# Autodesk Inventor assembly: 000-dribl-v2
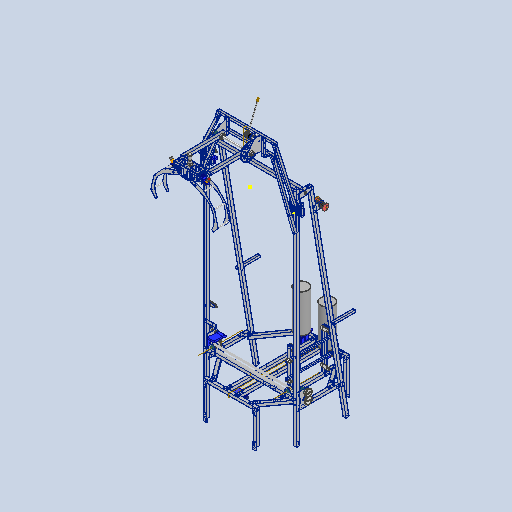
[picture p0: Inventor's stored thumbnail of the model, 512x512]
Saved by Autodesk Inventor 2025.2 (Build 292293000, 293)
## iProperties
Created: 2025-04-03
Part Number: 000-dribl-v2
Document SubType Name: Assembly
Designer: haruy
Author: haruy
## Documents named in this file (63)
- C:\Users\haruy\Documents\ロボコン\NHK2025\cad\nagahisa\dribl\000-dribl-v2.iam
- C:\Users\haruy\Documents\ロボコン\NHK2025\cad\nagahisa\dribl\dribl-v3-Sketch-Base.ipt
- C:\Users\haruy\Documents\ロボコン\NHK2025\cad\nagahisa\dribl\dribl-v1-Plate-5.ipt
- C:\Users\haruy\Documents\ロボコン\NHK2025\cad\nagahisa\dribl\dribl-v1-Plate-3.ipt
- C:\Users\haruy\Documents\ロボコン\NHK2025\cad\nagahisa\dribl\dribl-v1-Plate-4.ipt
- C:\Users\haruy\Documents\ロボコン\NHK2025\cad\nagahisa\dribl\dribl-v3-Plate-1.ipt
- C:\Users\haruy\Documents\ロボコン\NHK2025\cad\nagahisa\dribl\dribl-v3-Plate-2.ipt
- C:\Users\haruy\Documents\ロボコン\NHK2025\cad\nagahisa\dribl\dribl-v3-ASP-arm.ipt
- C:\Users\haruy\Documents\ロボコン\NHK2025\cad\nagahisa\dribl\dribl-v1-Shaft-spesa-57.ipt
- C:\Users\haruy\Documents\ロボコン\NHK2025\cad\nagahisa\dribl\dribl-v1-Plate-8.ipt
- C:\Users\haruy\Documents\ロボコン\NHK2025\cad\000_parts\モーター\robomaster\M2006 P36\RoboMaster M2006 P36\RoboMaster M2006 P36.ipt
- C:\Users\haruy\Documents\ロボコン\NHK2025\cad\nagahisa\dribl\dribl-v3-Plate-6.ipt
- C:\Users\haruy\Documents\ロボコン\NHK2025\cad\nagahisa\dribl\dribl-v3-Plate-7.ipt
- C:\Users\haruy\Documents\ロボコン\NHK2025\cad\nagahisa\dribl\dribl-v3-Plate-8.ipt
- C:\Users\haruy\Documents\ロボコン\NHK2025\cad\nagahisa\dribl\dribl-v3-Plate-9.ipt
- C:\Users\haruy\Documents\ロボコン\NHK2025\cad\nagahisa\dribl\dribl-v3-Plate-10.ipt
- C:\Users\haruy\Documents\ロボコン\NHK2025\cad\nagahisa\dribl\dribl-v3-Plate-11.ipt
- C:\Users\haruy\Documents\ロボコン\NHK2025\cad\nagahisa\dribl\dribl-v3-Plate-12.ipt
- C:\Users\haruy\Documents\ロボコン\NHK2025\cad\nagahisa\dribl\dribl-v1-Plate-14.ipt
- C:\Users\haruy\Documents\ロボコン\NHK2025\cad\nagahisa\dribl\dribl-v1-3DP-P-F.ipt
- C:\Users\haruy\Documents\ロボコン\NHK2025\cad\nagahisa\dribl\roller-Base-v1-petbottle.ipt
- C:\Users\haruy\Documents\ロボコン\NHK2025\cad\nagahisa\dribl\dribl-v3-Plate-13.ipt
- C:\Users\haruy\Documents\ロボコン\NHK2025\cad\nagahisa\dribl\dribl-v3-Plate-14.ipt
- C:\Users\haruy\Documents\ロボコン\NHK2025\cad\nagahisa\base_weel\base_weel-v2-Plate-8.ipt
- C:\Users\haruy\Documents\ロボコン\NHK2025\cad\nagahisa\dribl\dribl-v3-ASP-2.ipt
- C:\Users\haruy\Documents\ロボコン\NHK2025\cad\nagahisa\base_weel\base_weel-v2-POM-pc-F-1.ipt
- C:\Users\haruy\Documents\ロボコン\NHK2025\cad\nagahisa\base_weel\base_weel-v2-POM-pc-F-2.ipt
- C:\Users\haruy\Documents\ロボコン\NHK2025\cad\nagahisa\dribl\dribl-v3-Plate-15.ipt
- C:\Users\haruy\Documents\ロボコン\NHK2025\cad\nagahisa\dribl\dribl-v1-Plate-13.ipt
- C:\Users\haruy\Documents\ロボコン\NHK2025\cad\000_parts\回路関連\EMO\emo_sa.ipt
- C:\Users\haruy\Documents\ロボコン\NHK2025\cad\nagahisa\dribl\dribl-v1-Plate-12.ipt
- C:\Users\haruy\Documents\ロボコン\NHK2025\cad\000_parts\センサー\VX-012-1A3\VX-012-1A3\VX-012-1A3.iam
- C:\Users\haruy\Documents\ロボコン\NHK2025\cad\nagahisa\dribl\R2-Rzvector\TH22_bearing_12_18_19.5_sn.ipt
- C:\Users\haruy\Documents\ロボコン\NHK2025\cad\nagahisa\dribl\SCSNAJ12-16b.ipt
- C:\Users\haruy\Documents\ロボコン\NHK2025\cad\nagahisa\dribl\dribl-v1-Shaft-2.ipt
- C:\Users\haruy\Documents\ロボコン\NHK2025\cad\nagahisa\dribl\dribl-v3-3DP-2.ipt
- C:\Users\haruy\Documents\ロボコン\NHK2025\cad\000_parts\センサー\realsense\D435i_Solid.ipt
- C:\Users\haruy\Documents\ロボコン\NHK2025\cad\nagahisa\dribl\R2-Rzvector\bear_f8_12_sa.ipt
- C:\Users\haruy\Documents\ロボコン\NHK2025\cad\nagahisa\dribl\R2-Rzvector\bear_10_15_sn.ipt
- C:\Users\haruy\Documents\ロボコン\NHK2025\cad\nagahisa\dribl\SCTW12.iam
- C:\Users\haruy\Documents\ロボコン\NHK2025\cad\nagahisa\base_weel\SCSWA8-8.iam
- C:\Users\haruy\Documents\ロボコン\NHK2025\cad\nagahisa\belt_liner\SSCSW10-10b.ipt
- C:\Users\haruy\Documents\ロボコン\NHK2025\cad\nagahisa\dribl\000-dribl-v2\デザイン アクセラレータ\平歯車1.iam
- C:\Users\haruy\Documents\ロボコン\NHK2025\cad\nagahisa\dribl\000-dribl-v2\デザイン アクセラレータ\平歯車2.iam
- C:\Users\haruy\Documents\ロボコン\NHK2025\cad\nagahisa\hand\grab\hand-grab-v5-Plate-6.ipt
- C:\Users\haruy\Documents\ロボコン\NHK2025\cad\nagahisa\hand\grab\hand-grab-v5-Plate-7.ipt
- C:\Users\haruy\Documents\ロボコン\NHK2025\cad\nagahisa\hand\grab\000-hand-grab-v5.iam
- C:\Users\haruy\Documents\ロボコン\NHK2025\cad\nagahisa\hand\grab\hand-grab-v5-ASP-1.ipt
- C:\Users\haruy\Documents\ロボコン\NHK2025\cad\nagahisa\dribl\SCSW12-10.iam
- C:\Users\haruy\Documents\ロボコン\NHK2025\cad\nagahisa\dribl\dribl-v4-Plate-1.ipt
- C:\Users\haruy\Documents\ロボコン\NHK2025\cad\nagahisa\dribl\dribl-v4-Plate-2.ipt
- C:\Users\haruy\Documents\ロボコン\NHK2025\cad\nagahisa\dribl\000-dribl-v2\デザイン アクセラレータ\歯付きベルト伝達2.iam
- C:\Users\haruy\Documents\ロボコン\NHK2025\cad\nagahisa\dribl\000-dribl-v2\デザイン アクセラレータ\平歯車3.iam
- C:\Users\haruy\Documents\ロボコン\NHK2025\cad\nagahisa\dribl\SCSW6-10b.ipt
- C:\Users\haruy\Documents\ロボコン\NHK2025\cad\nagahisa\dribl\dribl-v4-Plate-3.ipt
- C:\Users\haruy\Documents\ロボコン\NHK2025\cad\nagahisa\dribl\R2-Rzvector\RZvector-v1-Plate-B-F.ipt
- C:\Users\haruy\Documents\ロボコン\NHK2025\cad\nagahisa\dribl\dribl-v4-3DP-1.ipt
- C:\Users\haruy\Documents\ロボコン\NHK2025\cad\nagahisa\dribl\dribl-v4-Plate-4.ipt
- C:\Users\haruy\Documents\ロボコン\NHK2025\cad\nagahisa\dribl\dribl-v1-Shaft-4.ipt
- C:\Users\haruy\Documents\ロボコン\NHK2025\cad\nagahisa\dribl\dribl-v1-Shaft-6.ipt
- C:\Users\haruy\Documents\ロボコン\NHK2025\cad\nagahisa\dribl\SMB1_5-20_SMB1_5-20_On.iam
- C:\Users\haruy\Documents\ロボコン\NHK2025\cad\nagahisa\dribl\dribl-v1-Shaft-1.ipt
- C:\Users\haruy\Documents\ロボコン\NHK2025\cad\nagahisa\dribl\dribl-v4-3DP-2.ipt
## Components (125 placed, 60 different names)
1. dribl-v3-Sketch-Base:1 — 挿入:11, 挿入:13, 挿入:14, 挿入:15, 挿入:16, 挿入:17, 挿入:18, 挿入:19, 挿入:20, 挿入:21, 挿入:22, 挿入:23, 挿入:24, 挿入:25, 挿入:26, 挿入:27, 挿入:28, 挿入:29, 挿入:30, 挿入:31, 挿入:32, 挿入:33, 正接:1, 正接:2, 正接:3, 正接:4, 挿入:44, 挿入:45, 挿入:46, 挿入:47, 挿入:48, 挿入:49, 挿入:50, 挿入:51, 挿入:52, 挿入:53, 挿入:56, 挿入:57, 挿入:58, 挿入:59, 挿入:60, 挿入:61, 挿入:62, 挿入:63, 挿入:64, 挿入:65, 挿入:70, 挿入:71, 挿入:72, 挿入:73, 挿入:74, 挿入:75, 挿入:76, 挿入:77, 挿入:78, 挿入:79, 挿入:80, 挿入:81, 挿入:82, 挿入:83, 挿入:84, 挿入:85, 挿入:90, 挿入:91, 挿入:92, 挿入:93, 挿入:94, 挿入:95, 挿入:96, 挿入:97, メイト:4, メイト:6, 挿入:102, 挿入:103, 挿入:104, 挿入:105, 挿入:106, 挿入:107, 挿入:108, 挿入:109, 挿入:128, 挿入:129, 挿入:130, 挿入:131, 挿入:132, 挿入:133, 挿入:134, 挿入:135, フラッシュ:1, 挿入:163, 挿入:164, 挿入:221, 挿入:225, 挿入:233, 挿入:234, 挿入:235, 挿入:236, 挿入:252, 挿入:253, メイト:16, メイト:17, 挿入:254, 挿入:255, 挿入:263, 挿入:264
2. dribl-v1-Plate-5:1 — 挿入:13, 挿入:173, 挿入:175, 挿入:264, 挿入:266, 挿入:267
3. dribl-v1-Plate-5:2 — 挿入:11, 挿入:174, 挿入:176, 挿入:263, 角度:1
4. dribl-v1-Plate-3:1 — 挿入:14, 挿入:15, 挿入:167, 挿入:183
5. dribl-v1-Plate-4:1 — 挿入:16, 挿入:17, 挿入:168
6. dribl-v3-Plate-1:1 — 挿入:18, 挿入:19, 挿入:172
7. dribl-v3-Plate-1:2 — 挿入:20, 挿入:21, 挿入:171
8. dribl-v3-Plate-1:3 — 挿入:22, 挿入:23, 挿入:170
9. dribl-v3-Plate-1:4 — 挿入:24, 挿入:25, 挿入:169
10. dribl-v3-Plate-2:1 — 挿入:26, 挿入:27, 挿入:179
11. dribl-v3-Plate-2:2 — 挿入:28, 挿入:29, 挿入:180
12. dribl-v3-Plate-2:3 — 挿入:32, 挿入:33, 挿入:177
13. dribl-v3-Plate-2:4 — 挿入:30, 挿入:31, 挿入:178
14. dribl-v3-ASP-arm:1 — 正接:1, 正接:2, 正接:3, 正接:4, 挿入:202, 挿入:203, 挿入:204, 挿入:205, 挿入:212, 挿入:213, 挿入:214, 挿入:215, 挿入:216, 挿入:217, 挿入:218, 挿入:219, 挿入:237, 挿入:238, 挿入:239, 挿入:240, 挿入:241, 挿入:268, 挿入:269
15. dribl-v1-Shaft-spesa-57:1 — 挿入:41, 挿入:206
16. dribl-v1-Shaft-spesa-57:2 — 挿入:208
17. dribl-v1-Shaft-spesa-57:3 — 挿入:42, 挿入:207
18. dribl-v1-Plate-8:1 — 挿入:41, 挿入:42, 挿入:43, 挿入:208
19. RoboMaster M2006 P36:1 — 挿入:43, メイト:15
20. dribl-v3-Plate-6:1 — 挿入:44, 挿入:45
21. dribl-v3-Plate-6:2 — 挿入:50, 挿入:51
22. dribl-v3-Plate-6:3 — 挿入:48, 挿入:49
23. dribl-v3-Plate-6:4 — 挿入:46, 挿入:47
24. dribl-v3-Plate-7:1 — 挿入:52, 挿入:53
25. dribl-v3-Plate-7:4 — 挿入:56, 挿入:57
26. dribl-v3-Plate-8:1 — 挿入:58, 挿入:59
27. dribl-v3-Plate-8:2 — 挿入:60, 挿入:61
28. dribl-v3-Plate-9:1 — 挿入:62, 挿入:63
29. dribl-v3-Plate-9:3 — 挿入:64, 挿入:65
30. dribl-v3-Plate-10:1 — 挿入:72, 挿入:73
31. dribl-v3-Plate-10:2 — 挿入:74, 挿入:75
32. dribl-v3-Plate-10:3 — 挿入:70, 挿入:71
33. dribl-v3-Plate-10:4 — 挿入:76, 挿入:77
34. dribl-v3-Plate-11:1 — 挿入:78, 挿入:79
35. dribl-v3-Plate-11:2 — 挿入:82, 挿入:83
36. dribl-v3-Plate-11:3 — 挿入:80, 挿入:81
37. dribl-v3-Plate-11:4 — 挿入:84, 挿入:85
38. dribl-v3-Plate-12:1 — 挿入:90, 挿入:91
39. dribl-v3-Plate-12:2 — 挿入:92, 挿入:93
40. dribl-v1-Plate-14:1 — 挿入:96, 挿入:97
41. dribl-v1-Plate-14:2 — 挿入:94, 挿入:95
42. dribl-v1-3DP-P-F:1 — 挿入:100, メイト:6, メイト:16
43. roller-Base-v1-petbottle:1 — 挿入:100
44. dribl-v1-3DP-P-F:2 — メイト:4, 挿入:101, メイト:17
45. roller-Base-v1-petbottle:2 — 挿入:101
46. dribl-v3-Plate-13:1 — 挿入:102, 挿入:103
47. dribl-v3-Plate-14:1 — 挿入:104, 挿入:105
48. base_weel-v2-Plate-8:1 — 挿入:106, 挿入:107, 挿入:110, 挿入:111
49. base_weel-v2-Plate-8:2 — 挿入:108, 挿入:109
50. dribl-v3-ASP-2:1 — 挿入:110, 挿入:111, 挿入:112, 挿入:113, 挿入:114, 挿入:115, 挿入:116, 挿入:117, 挿入:118, 挿入:119, 挿入:120, 挿入:121, 挿入:122, 挿入:123, 挿入:124, 挿入:125, 挿入:126, 挿入:127
51. base_weel-v2-POM-pc-F-1:1 — 挿入:112, 挿入:113
52. base_weel-v2-POM-pc-F-1:2 — 挿入:114, 挿入:115
53. base_weel-v2-POM-pc-F-2:1 — 挿入:118, 挿入:119
54. base_weel-v2-POM-pc-F-2:2 — 挿入:116, 挿入:117
55. base_weel-v2-POM-pc-F-2:3 — 挿入:122, 挿入:123
56. base_weel-v2-POM-pc-F-2:4 — 挿入:120, 挿入:121
57. base_weel-v2-POM-pc-F-1:3 — 挿入:126, 挿入:127
58. base_weel-v2-POM-pc-F-1:4 — 挿入:124, 挿入:125
59. dribl-v3-Plate-15:1 — 挿入:128, 挿入:129
60. dribl-v3-Plate-15:2 — 挿入:130, 挿入:131
61. dribl-v3-Plate-11:7 — 挿入:132, 挿入:133
62. dribl-v1-Plate-13:1 — 挿入:134, 挿入:135, 挿入:136
63. emo_sa:1 — 挿入:136
64. VX-012-1A3:1 [sub-assembly] — 挿入:223, 挿入:224
65. TH22_bearing_12_18_19.5_sn:1 — 挿入:160, 挿入:210
66. TH22_bearing_12_18_19.5_sn:2 — 挿入:194, 挿入:209
67. SCSNAJ12-16b:1 — 挿入:194
68. SCSNAJ12-16b:2 — 挿入:160, 挿入:195
69. dribl-v1-Shaft-2:1 — 挿入:195, メイト:13
70. dribl-v3-3DP-2:1 — 挿入:163, 挿入:164, 挿入:165, 挿入:166
71. D435i_Solid:1 — 挿入:165, 挿入:166
72. TH22_bearing_12_18_19.5_sn:3 — 挿入:167, 挿入:184
73. TH22_bearing_12_18_19.5_sn:4 — 挿入:168
74. TH22_bearing_12_18_19.5_sn:5 — 挿入:170
75. TH22_bearing_12_18_19.5_sn:6 — 挿入:169, フラッシュ:2
76. TH22_bearing_12_18_19.5_sn:7 — 挿入:171
77. TH22_bearing_12_18_19.5_sn:8 — 挿入:172, 挿入:261
78. TH22_bearing_12_18_19.5_sn:9 — 挿入:173
79. TH22_bearing_12_18_19.5_sn:10 — 挿入:174, 挿入:181
80. bear_f8_12_sa:1 — 挿入:175, 挿入:258
81. bear_f8_12_sa:2 — 挿入:176, 挿入:182
82. bear_10_15_sn:3 — 挿入:178
83. bear_10_15_sn:4 — 挿入:177
84. bear_10_15_sn:5 — 挿入:179
85. bear_10_15_sn:6 — 挿入:180
86. SCTW12:1 [sub-assembly] — 挿入:181, メイト:20
87. SCSWA8-8:1 [sub-assembly] — 挿入:182, メイト:18, メイト:19
88. SSCSW10-10b:1 — 挿入:183, メイト:9
89. SCTW12:2 [sub-assembly] — 挿入:184, メイト:7, メイト:8
90. 平歯車:1 [sub-assembly] — メイト:7, メイト:8, メイト:9
91. 平歯車:2 [sub-assembly] — メイト:18, メイト:19, メイト:20
92. hand-grab-v5-Plate-6:1 — 挿入:202, 挿入:203, 挿入:206, 挿入:207, 挿入:210, 挿入:211
93. hand-grab-v5-Plate-7:1 — 挿入:204, 挿入:205, 挿入:209
94. 000-hand-grab-v5:1 [sub-assembly] — 挿入:196, 挿入:197, 挿入:198, 挿入:199
95. hand-grab-v5-ASP-1:1 — 挿入:196, 挿入:197, 挿入:200
96. hand-grab-v5-ASP-1:2 — 挿入:198, 挿入:199, 挿入:201, 挿入:211, メイト:14
97. SCSW12-10:1 [sub-assembly] — 挿入:201
98. SCSW12-10:2 [sub-assembly] — 挿入:200
99. dribl-v4-Plate-1:1 — 挿入:212, 挿入:213
100. dribl-v4-Plate-1:2 — 挿入:214, 挿入:215
101. dribl-v4-Plate-2:1 — 挿入:216, 挿入:217
102. dribl-v4-Plate-2:2 — 挿入:218, 挿入:219
103. 歯付きベルト伝達:1 [sub-assembly]
104. 平歯車:3 [sub-assembly] — メイト:13, メイト:14, メイト:15, 挿入:220
105. SCSW6-10b:1 — 挿入:220
106. dribl-v1-Plate-12:2 — 挿入:221, 挿入:223, 挿入:224, 挿入:233
107. dribl-v1-Plate-12:3 — 挿入:225, 挿入:227, 挿入:228, 挿入:234
108. VX-012-1A3:3 [sub-assembly] — 挿入:227, 挿入:228
109. dribl-v1-Plate-12:4 — 挿入:231, 挿入:232, 挿入:235, 挿入:236
110. VX-012-1A3:4 [sub-assembly] — 挿入:231, 挿入:232
111. dribl-v4-Plate-3:1 — 挿入:240, 挿入:241, 挿入:242, 挿入:243, 挿入:244, 挿入:245
112. dribl-v4-Plate-3:2 — 挿入:237, 挿入:238, 挿入:239, 挿入:246, 挿入:247, 挿入:248, 挿入:249
113. RZvector-v1-Plate-B-F:1 — 挿入:242, 挿入:243
114. RZvector-v1-Plate-B-F:2 — 挿入:244, 挿入:245
115. RZvector-v1-Plate-B-F:3 — 挿入:246, 挿入:247
116. RZvector-v1-Plate-B-F:4 — 挿入:248, 挿入:249
117. dribl-v4-3DP-1:1 — 挿入:268, 挿入:269
118. dribl-v4-Plate-4:1 — 挿入:252, 挿入:253
119. dribl-v1-Plate-12:5 — 挿入:254, 挿入:255, 挿入:256, 挿入:257
120. VX-012-1A3:5 [sub-assembly] — 挿入:256, 挿入:257
121. dribl-v1-Shaft-4:1 — 挿入:258
122. dribl-v1-Shaft-6:1 — 挿入:265, 角度:1
123. SMB1_5-20_SMB1_5-20_On:1 [sub-assembly] — 挿入:262, 挿入:265
124. dribl-v1-Shaft-1:1 — 挿入:261, 挿入:262
125. dribl-v4-3DP-2:1 — 挿入:266, 挿入:267
## Relationships (217: Insert 197, Mate 13, Tangent 4, Flush 2, Angle 1)
- 挿入:11 [Insert]: dribl-v3-Sketch-Base:1 ↔ dribl-v1-Plate-5:2
- 挿入:13 [Insert]: dribl-v3-Sketch-Base:1 ↔ dribl-v1-Plate-5:1
- 挿入:14 [Insert]: dribl-v3-Sketch-Base:1 ↔ dribl-v1-Plate-3:1
- 挿入:15 [Insert]: dribl-v3-Sketch-Base:1 ↔ dribl-v1-Plate-3:1
- 挿入:16 [Insert]: dribl-v3-Sketch-Base:1 ↔ dribl-v1-Plate-4:1
- 挿入:17 [Insert]: dribl-v3-Sketch-Base:1 ↔ dribl-v1-Plate-4:1
- 挿入:18 [Insert]: dribl-v3-Sketch-Base:1 ↔ dribl-v3-Plate-1:1
- 挿入:19 [Insert]: dribl-v3-Sketch-Base:1 ↔ dribl-v3-Plate-1:1
- 挿入:20 [Insert]: dribl-v3-Sketch-Base:1 ↔ dribl-v3-Plate-1:2
- 挿入:21 [Insert]: dribl-v3-Sketch-Base:1 ↔ dribl-v3-Plate-1:2
- 挿入:22 [Insert]: dribl-v3-Sketch-Base:1 ↔ dribl-v3-Plate-1:3
- 挿入:23 [Insert]: dribl-v3-Sketch-Base:1 ↔ dribl-v3-Plate-1:3
- 挿入:24 [Insert]: dribl-v3-Sketch-Base:1 ↔ dribl-v3-Plate-1:4
- 挿入:25 [Insert]: dribl-v3-Sketch-Base:1 ↔ dribl-v3-Plate-1:4
- 挿入:26 [Insert]: dribl-v3-Sketch-Base:1 ↔ dribl-v3-Plate-2:1
- 挿入:27 [Insert]: dribl-v3-Sketch-Base:1 ↔ dribl-v3-Plate-2:1
- 挿入:28 [Insert]: dribl-v3-Sketch-Base:1 ↔ dribl-v3-Plate-2:2
- 挿入:29 [Insert]: dribl-v3-Sketch-Base:1 ↔ dribl-v3-Plate-2:2
- 挿入:30 [Insert]: dribl-v3-Sketch-Base:1 ↔ dribl-v3-Plate-2:4
- 挿入:31 [Insert]: dribl-v3-Sketch-Base:1 ↔ dribl-v3-Plate-2:4
- 挿入:32 [Insert]: dribl-v3-Sketch-Base:1 ↔ dribl-v3-Plate-2:3
- 挿入:33 [Insert]: dribl-v3-Sketch-Base:1 ↔ dribl-v3-Plate-2:3
- 正接:1 [Tangent]: dribl-v3-Sketch-Base:1 ↔ dribl-v3-ASP-arm:1
- 正接:2 [Tangent]: dribl-v3-Sketch-Base:1 ↔ dribl-v3-ASP-arm:1
- 正接:3 [Tangent]: dribl-v3-Sketch-Base:1 ↔ dribl-v3-ASP-arm:1
- 正接:4 [Tangent]: dribl-v3-Sketch-Base:1 ↔ dribl-v3-ASP-arm:1
- 挿入:41 [Insert]: dribl-v1-Shaft-spesa-57:1 ↔ dribl-v1-Plate-8:1
- 挿入:42 [Insert]: dribl-v1-Shaft-spesa-57:3 ↔ dribl-v1-Plate-8:1
- 挿入:43 [Insert]: dribl-v1-Plate-8:1 ↔ RoboMaster M2006 P36:1
- 挿入:44 [Insert]: dribl-v3-Sketch-Base:1 ↔ dribl-v3-Plate-6:1
- 挿入:45 [Insert]: dribl-v3-Sketch-Base:1 ↔ dribl-v3-Plate-6:1
- 挿入:46 [Insert]: dribl-v3-Sketch-Base:1 ↔ dribl-v3-Plate-6:4
- 挿入:47 [Insert]: dribl-v3-Sketch-Base:1 ↔ dribl-v3-Plate-6:4
- 挿入:48 [Insert]: dribl-v3-Sketch-Base:1 ↔ dribl-v3-Plate-6:3
- 挿入:49 [Insert]: dribl-v3-Sketch-Base:1 ↔ dribl-v3-Plate-6:3
- 挿入:50 [Insert]: dribl-v3-Sketch-Base:1 ↔ dribl-v3-Plate-6:2
- 挿入:51 [Insert]: dribl-v3-Sketch-Base:1 ↔ dribl-v3-Plate-6:2
- 挿入:52 [Insert]: dribl-v3-Sketch-Base:1 ↔ dribl-v3-Plate-7:1
- 挿入:53 [Insert]: dribl-v3-Sketch-Base:1 ↔ dribl-v3-Plate-7:1
- 挿入:56 [Insert]: dribl-v3-Sketch-Base:1 ↔ dribl-v3-Plate-7:4
- 挿入:57 [Insert]: dribl-v3-Sketch-Base:1 ↔ dribl-v3-Plate-7:4
- 挿入:58 [Insert]: dribl-v3-Sketch-Base:1 ↔ dribl-v3-Plate-8:1
- 挿入:59 [Insert]: dribl-v3-Sketch-Base:1 ↔ dribl-v3-Plate-8:1
- 挿入:60 [Insert]: dribl-v3-Sketch-Base:1 ↔ dribl-v3-Plate-8:2
- 挿入:61 [Insert]: dribl-v3-Sketch-Base:1 ↔ dribl-v3-Plate-8:2
- 挿入:62 [Insert]: dribl-v3-Sketch-Base:1 ↔ dribl-v3-Plate-9:1
- 挿入:63 [Insert]: dribl-v3-Sketch-Base:1 ↔ dribl-v3-Plate-9:1
- 挿入:64 [Insert]: dribl-v3-Sketch-Base:1 ↔ dribl-v3-Plate-9:3
- 挿入:65 [Insert]: dribl-v3-Sketch-Base:1 ↔ dribl-v3-Plate-9:3
- 挿入:70 [Insert]: dribl-v3-Sketch-Base:1 ↔ dribl-v3-Plate-10:3
- 挿入:71 [Insert]: dribl-v3-Sketch-Base:1 ↔ dribl-v3-Plate-10:3
- 挿入:72 [Insert]: dribl-v3-Sketch-Base:1 ↔ dribl-v3-Plate-10:1
- 挿入:73 [Insert]: dribl-v3-Sketch-Base:1 ↔ dribl-v3-Plate-10:1
- 挿入:74 [Insert]: dribl-v3-Sketch-Base:1 ↔ dribl-v3-Plate-10:2
- 挿入:75 [Insert]: dribl-v3-Sketch-Base:1 ↔ dribl-v3-Plate-10:2
- 挿入:76 [Insert]: dribl-v3-Sketch-Base:1 ↔ dribl-v3-Plate-10:4
- 挿入:77 [Insert]: dribl-v3-Sketch-Base:1 ↔ dribl-v3-Plate-10:4
- 挿入:78 [Insert]: dribl-v3-Sketch-Base:1 ↔ dribl-v3-Plate-11:1
- 挿入:79 [Insert]: dribl-v3-Sketch-Base:1 ↔ dribl-v3-Plate-11:1
- 挿入:80 [Insert]: dribl-v3-Sketch-Base:1 ↔ dribl-v3-Plate-11:3
- 挿入:81 [Insert]: dribl-v3-Sketch-Base:1 ↔ dribl-v3-Plate-11:3
- 挿入:82 [Insert]: dribl-v3-Sketch-Base:1 ↔ dribl-v3-Plate-11:2
- 挿入:83 [Insert]: dribl-v3-Sketch-Base:1 ↔ dribl-v3-Plate-11:2
- 挿入:84 [Insert]: dribl-v3-Sketch-Base:1 ↔ dribl-v3-Plate-11:4
- 挿入:85 [Insert]: dribl-v3-Sketch-Base:1 ↔ dribl-v3-Plate-11:4
- 挿入:90 [Insert]: dribl-v3-Sketch-Base:1 ↔ dribl-v3-Plate-12:1
- 挿入:91 [Insert]: dribl-v3-Sketch-Base:1 ↔ dribl-v3-Plate-12:1
- 挿入:92 [Insert]: dribl-v3-Sketch-Base:1 ↔ dribl-v3-Plate-12:2
- 挿入:93 [Insert]: dribl-v3-Sketch-Base:1 ↔ dribl-v3-Plate-12:2
- 挿入:94 [Insert]: dribl-v3-Sketch-Base:1 ↔ dribl-v1-Plate-14:2
- 挿入:95 [Insert]: dribl-v3-Sketch-Base:1 ↔ dribl-v1-Plate-14:2
- 挿入:96 [Insert]: dribl-v3-Sketch-Base:1 ↔ dribl-v1-Plate-14:1
- 挿入:97 [Insert]: dribl-v3-Sketch-Base:1 ↔ dribl-v1-Plate-14:1
- 挿入:100 [Insert]: dribl-v1-3DP-P-F:1 ↔ roller-Base-v1-petbottle:1
- メイト:4 [Mate]: dribl-v3-Sketch-Base:1 ↔ dribl-v1-3DP-P-F:2
- 挿入:101 [Insert]: dribl-v1-3DP-P-F:2 ↔ roller-Base-v1-petbottle:2
- メイト:6 [Mate]: dribl-v3-Sketch-Base:1 ↔ dribl-v1-3DP-P-F:1
- 挿入:102 [Insert]: dribl-v3-Sketch-Base:1 ↔ dribl-v3-Plate-13:1
- 挿入:103 [Insert]: dribl-v3-Sketch-Base:1 ↔ dribl-v3-Plate-13:1
- 挿入:104 [Insert]: dribl-v3-Sketch-Base:1 ↔ dribl-v3-Plate-14:1
- 挿入:105 [Insert]: dribl-v3-Sketch-Base:1 ↔ dribl-v3-Plate-14:1
- 挿入:106 [Insert]: dribl-v3-Sketch-Base:1 ↔ base_weel-v2-Plate-8:1
- 挿入:107 [Insert]: dribl-v3-Sketch-Base:1 ↔ base_weel-v2-Plate-8:1
- 挿入:108 [Insert]: dribl-v3-Sketch-Base:1 ↔ base_weel-v2-Plate-8:2
- 挿入:109 [Insert]: dribl-v3-Sketch-Base:1 ↔ base_weel-v2-Plate-8:2
- 挿入:110 [Insert]: base_weel-v2-Plate-8:1 ↔ dribl-v3-ASP-2:1
- 挿入:111 [Insert]: base_weel-v2-Plate-8:1 ↔ dribl-v3-ASP-2:1
- 挿入:112 [Insert]: dribl-v3-ASP-2:1 ↔ base_weel-v2-POM-pc-F-1:1
- 挿入:113 [Insert]: dribl-v3-ASP-2:1 ↔ base_weel-v2-POM-pc-F-1:1
- 挿入:114 [Insert]: dribl-v3-ASP-2:1 ↔ base_weel-v2-POM-pc-F-1:2
- 挿入:115 [Insert]: dribl-v3-ASP-2:1 ↔ base_weel-v2-POM-pc-F-1:2
- 挿入:116 [Insert]: dribl-v3-ASP-2:1 ↔ base_weel-v2-POM-pc-F-2:2
- 挿入:117 [Insert]: dribl-v3-ASP-2:1 ↔ base_weel-v2-POM-pc-F-2:2
- 挿入:118 [Insert]: dribl-v3-ASP-2:1 ↔ base_weel-v2-POM-pc-F-2:1
- 挿入:119 [Insert]: dribl-v3-ASP-2:1 ↔ base_weel-v2-POM-pc-F-2:1
- 挿入:120 [Insert]: dribl-v3-ASP-2:1 ↔ base_weel-v2-POM-pc-F-2:4
- 挿入:121 [Insert]: dribl-v3-ASP-2:1 ↔ base_weel-v2-POM-pc-F-2:4
- 挿入:122 [Insert]: dribl-v3-ASP-2:1 ↔ base_weel-v2-POM-pc-F-2:3
- 挿入:123 [Insert]: dribl-v3-ASP-2:1 ↔ base_weel-v2-POM-pc-F-2:3
- 挿入:124 [Insert]: dribl-v3-ASP-2:1 ↔ base_weel-v2-POM-pc-F-1:4
- 挿入:125 [Insert]: dribl-v3-ASP-2:1 ↔ base_weel-v2-POM-pc-F-1:4
- 挿入:126 [Insert]: dribl-v3-ASP-2:1 ↔ base_weel-v2-POM-pc-F-1:3
- 挿入:127 [Insert]: dribl-v3-ASP-2:1 ↔ base_weel-v2-POM-pc-F-1:3
- 挿入:128 [Insert]: dribl-v3-Sketch-Base:1 ↔ dribl-v3-Plate-15:1
- 挿入:129 [Insert]: dribl-v3-Sketch-Base:1 ↔ dribl-v3-Plate-15:1
- 挿入:130 [Insert]: dribl-v3-Sketch-Base:1 ↔ dribl-v3-Plate-15:2
- 挿入:131 [Insert]: dribl-v3-Sketch-Base:1 ↔ dribl-v3-Plate-15:2
- 挿入:132 [Insert]: dribl-v3-Sketch-Base:1 ↔ dribl-v3-Plate-11:7
- 挿入:133 [Insert]: dribl-v3-Sketch-Base:1 ↔ dribl-v3-Plate-11:7
- 挿入:134 [Insert]: dribl-v3-Sketch-Base:1 ↔ dribl-v1-Plate-13:1
- 挿入:135 [Insert]: dribl-v3-Sketch-Base:1 ↔ dribl-v1-Plate-13:1
- 挿入:136 [Insert]: dribl-v1-Plate-13:1 ↔ emo_sa:1
- フラッシュ:1 [Flush] (-10 mm): dribl-v3-Sketch-Base:1
- 挿入:160 [Insert]: TH22_bearing_12_18_19.5_sn:1 ↔ SCSNAJ12-16b:2
- 挿入:163 [Insert]: dribl-v3-Sketch-Base:1 ↔ dribl-v3-3DP-2:1
- 挿入:164 [Insert]: dribl-v3-Sketch-Base:1 ↔ dribl-v3-3DP-2:1
- 挿入:165 [Insert]: dribl-v3-3DP-2:1 ↔ D435i_Solid:1
- 挿入:166 [Insert]: dribl-v3-3DP-2:1 ↔ D435i_Solid:1
- 挿入:167 [Insert]: dribl-v1-Plate-3:1 ↔ TH22_bearing_12_18_19.5_sn:3
- 挿入:168 [Insert]: dribl-v1-Plate-4:1 ↔ TH22_bearing_12_18_19.5_sn:4
- 挿入:169 [Insert]: dribl-v3-Plate-1:4 ↔ TH22_bearing_12_18_19.5_sn:6
- 挿入:170 [Insert]: dribl-v3-Plate-1:3 ↔ TH22_bearing_12_18_19.5_sn:5
- 挿入:171 [Insert]: dribl-v3-Plate-1:2 ↔ TH22_bearing_12_18_19.5_sn:7
- 挿入:172 [Insert]: dribl-v3-Plate-1:1 ↔ TH22_bearing_12_18_19.5_sn:8
- 挿入:173 [Insert]: dribl-v1-Plate-5:1 ↔ TH22_bearing_12_18_19.5_sn:9
- 挿入:174 [Insert]: dribl-v1-Plate-5:2 ↔ TH22_bearing_12_18_19.5_sn:10
- 挿入:175 [Insert]: dribl-v1-Plate-5:1 ↔ bear_f8_12_sa:1
- 挿入:176 [Insert]: dribl-v1-Plate-5:2 ↔ bear_f8_12_sa:2
- 挿入:177 [Insert]: dribl-v3-Plate-2:3 ↔ bear_10_15_sn:4
- 挿入:178 [Insert]: dribl-v3-Plate-2:4 ↔ bear_10_15_sn:3
- 挿入:179 [Insert]: dribl-v3-Plate-2:1 ↔ bear_10_15_sn:5
- 挿入:180 [Insert]: dribl-v3-Plate-2:2 ↔ bear_10_15_sn:6
- 挿入:181 [Insert] (5 mm): TH22_bearing_12_18_19.5_sn:10 ↔ SCTW12:1
- 挿入:182 [Insert] (9.3 mm): bear_f8_12_sa:2 ↔ SCSWA8-8:1
- 挿入:183 [Insert] (7 mm): dribl-v1-Plate-3:1 ↔ SSCSW10-10b:1
- 挿入:184 [Insert] (4 mm): TH22_bearing_12_18_19.5_sn:3 ↔ SCTW12:2
- メイト:7 [Mate]: SCTW12:2 ↔ 平歯車:1
- メイト:8 [Mate]: SCTW12:2 ↔ 平歯車:1
- メイト:9 [Mate]: SSCSW10-10b:1 ↔ 平歯車:1
- 挿入:194 [Insert]: TH22_bearing_12_18_19.5_sn:2 ↔ SCSNAJ12-16b:1
- 挿入:195 [Insert]: SCSNAJ12-16b:2 ↔ dribl-v1-Shaft-2:1
- 挿入:196 [Insert]: 000-hand-grab-v5:1 ↔ hand-grab-v5-ASP-1:1
- 挿入:197 [Insert]: 000-hand-grab-v5:1 ↔ hand-grab-v5-ASP-1:1
- 挿入:198 [Insert]: 000-hand-grab-v5:1 ↔ hand-grab-v5-ASP-1:2
- 挿入:199 [Insert]: 000-hand-grab-v5:1 ↔ hand-grab-v5-ASP-1:2
- 挿入:200 [Insert]: hand-grab-v5-ASP-1:1 ↔ SCSW12-10:2
- 挿入:201 [Insert]: hand-grab-v5-ASP-1:2 ↔ SCSW12-10:1
- 挿入:202 [Insert]: dribl-v3-ASP-arm:1 ↔ hand-grab-v5-Plate-6:1
- 挿入:203 [Insert]: dribl-v3-ASP-arm:1 ↔ hand-grab-v5-Plate-6:1
- 挿入:204 [Insert]: dribl-v3-ASP-arm:1 ↔ hand-grab-v5-Plate-7:1
- 挿入:205 [Insert]: dribl-v3-ASP-arm:1 ↔ hand-grab-v5-Plate-7:1
- 挿入:206 [Insert]: dribl-v1-Shaft-spesa-57:1 ↔ hand-grab-v5-Plate-6:1
- 挿入:207 [Insert]: dribl-v1-Shaft-spesa-57:3 ↔ hand-grab-v5-Plate-6:1
- 挿入:208 [Insert]: dribl-v1-Shaft-spesa-57:2 ↔ dribl-v1-Plate-8:1
- 挿入:209 [Insert]: TH22_bearing_12_18_19.5_sn:2 ↔ hand-grab-v5-Plate-7:1
- 挿入:210 [Insert]: TH22_bearing_12_18_19.5_sn:1 ↔ hand-grab-v5-Plate-6:1
- 挿入:211 [Insert] (13 mm): hand-grab-v5-Plate-6:1 ↔ hand-grab-v5-ASP-1:2
- 挿入:212 [Insert]: dribl-v3-ASP-arm:1 ↔ dribl-v4-Plate-1:1
- 挿入:213 [Insert]: dribl-v3-ASP-arm:1 ↔ dribl-v4-Plate-1:1
- 挿入:214 [Insert]: dribl-v3-ASP-arm:1 ↔ dribl-v4-Plate-1:2
- 挿入:215 [Insert]: dribl-v3-ASP-arm:1 ↔ dribl-v4-Plate-1:2
- 挿入:216 [Insert]: dribl-v3-ASP-arm:1 ↔ dribl-v4-Plate-2:1
- 挿入:217 [Insert]: dribl-v3-ASP-arm:1 ↔ dribl-v4-Plate-2:1
- 挿入:218 [Insert]: dribl-v3-ASP-arm:1 ↔ dribl-v4-Plate-2:2
- 挿入:219 [Insert]: dribl-v3-ASP-arm:1 ↔ dribl-v4-Plate-2:2
- フラッシュ:2 [Flush] (9 mm): TH22_bearing_12_18_19.5_sn:6
- メイト:13 [Mate]: dribl-v1-Shaft-2:1 ↔ 平歯車:3
- メイト:14 [Mate]: hand-grab-v5-ASP-1:2 ↔ 平歯車:3
- メイト:15 [Mate]: RoboMaster M2006 P36:1 ↔ 平歯車:3
- 挿入:220 [Insert]: 平歯車:3 ↔ SCSW6-10b:1
- 挿入:221 [Insert]: dribl-v3-Sketch-Base:1 ↔ dribl-v1-Plate-12:2
- 挿入:223 [Insert]: VX-012-1A3:1 ↔ dribl-v1-Plate-12:2
- 挿入:224 [Insert]: VX-012-1A3:1 ↔ dribl-v1-Plate-12:2
- 挿入:225 [Insert]: dribl-v3-Sketch-Base:1 ↔ dribl-v1-Plate-12:3
- 挿入:227 [Insert]: dribl-v1-Plate-12:3 ↔ VX-012-1A3:3
- 挿入:228 [Insert]: dribl-v1-Plate-12:3 ↔ VX-012-1A3:3
- 挿入:231 [Insert]: dribl-v1-Plate-12:4 ↔ VX-012-1A3:4
- 挿入:232 [Insert]: dribl-v1-Plate-12:4 ↔ VX-012-1A3:4
- 挿入:233 [Insert]: dribl-v3-Sketch-Base:1 ↔ dribl-v1-Plate-12:2
- 挿入:234 [Insert]: dribl-v3-Sketch-Base:1 ↔ dribl-v1-Plate-12:3
- 挿入:235 [Insert]: dribl-v3-Sketch-Base:1 ↔ dribl-v1-Plate-12:4
- 挿入:236 [Insert]: dribl-v3-Sketch-Base:1 ↔ dribl-v1-Plate-12:4
- 挿入:237 [Insert]: dribl-v3-ASP-arm:1 ↔ dribl-v4-Plate-3:2
- 挿入:238 [Insert]: dribl-v3-ASP-arm:1 ↔ dribl-v4-Plate-3:2
- 挿入:239 [Insert]: dribl-v3-ASP-arm:1 ↔ dribl-v4-Plate-3:2
- 挿入:240 [Insert]: dribl-v3-ASP-arm:1 ↔ dribl-v4-Plate-3:1
- 挿入:241 [Insert]: dribl-v3-ASP-arm:1 ↔ dribl-v4-Plate-3:1
- 挿入:242 [Insert]: dribl-v4-Plate-3:1 ↔ RZvector-v1-Plate-B-F:1
- 挿入:243 [Insert]: dribl-v4-Plate-3:1 ↔ RZvector-v1-Plate-B-F:1
- 挿入:244 [Insert]: dribl-v4-Plate-3:1 ↔ RZvector-v1-Plate-B-F:2
- 挿入:245 [Insert]: dribl-v4-Plate-3:1 ↔ RZvector-v1-Plate-B-F:2
- 挿入:246 [Insert]: dribl-v4-Plate-3:2 ↔ RZvector-v1-Plate-B-F:3
- 挿入:247 [Insert]: dribl-v4-Plate-3:2 ↔ RZvector-v1-Plate-B-F:3
- 挿入:248 [Insert]: dribl-v4-Plate-3:2 ↔ RZvector-v1-Plate-B-F:4
- 挿入:249 [Insert]: dribl-v4-Plate-3:2 ↔ RZvector-v1-Plate-B-F:4
- 挿入:252 [Insert]: dribl-v3-Sketch-Base:1 ↔ dribl-v4-Plate-4:1
- 挿入:253 [Insert]: dribl-v3-Sketch-Base:1 ↔ dribl-v4-Plate-4:1
- メイト:16 [Mate]: dribl-v3-Sketch-Base:1 ↔ dribl-v1-3DP-P-F:1
- メイト:17 [Mate]: dribl-v3-Sketch-Base:1 ↔ dribl-v1-3DP-P-F:2
- 挿入:254 [Insert]: dribl-v3-Sketch-Base:1 ↔ dribl-v1-Plate-12:5
- 挿入:255 [Insert]: dribl-v3-Sketch-Base:1 ↔ dribl-v1-Plate-12:5
- 挿入:256 [Insert]: dribl-v1-Plate-12:5 ↔ VX-012-1A3:5
- 挿入:257 [Insert]: dribl-v1-Plate-12:5 ↔ VX-012-1A3:5
- 挿入:258 [Insert]: bear_f8_12_sa:1 ↔ dribl-v1-Shaft-4:1
- 挿入:261 [Insert]: TH22_bearing_12_18_19.5_sn:8 ↔ dribl-v1-Shaft-1:1
- 挿入:262 [Insert]: SMB1_5-20_SMB1_5-20_On:1 ↔ dribl-v1-Shaft-1:1
- 挿入:263 [Insert]: dribl-v3-Sketch-Base:1 ↔ dribl-v1-Plate-5:2
- 挿入:264 [Insert]: dribl-v3-Sketch-Base:1 ↔ dribl-v1-Plate-5:1
- 挿入:265 [Insert]: dribl-v1-Shaft-6:1 ↔ SMB1_5-20_SMB1_5-20_On:1
- 角度:1 [Angle] (0 deg): dribl-v1-Plate-5:2 ↔ dribl-v1-Shaft-6:1
- メイト:18 [Mate]: SCSWA8-8:1 ↔ 平歯車:2
- メイト:19 [Mate]: SCSWA8-8:1 ↔ 平歯車:2
- メイト:20 [Mate]: SCTW12:1 ↔ 平歯車:2
- 挿入:266 [Insert]: dribl-v1-Plate-5:1 ↔ dribl-v4-3DP-2:1
- 挿入:267 [Insert]: dribl-v1-Plate-5:1 ↔ dribl-v4-3DP-2:1
- 挿入:268 [Insert]: dribl-v3-ASP-arm:1 ↔ dribl-v4-3DP-1:1
- 挿入:269 [Insert]: dribl-v3-ASP-arm:1 ↔ dribl-v4-3DP-1:1
